# Autodesk Inventor assembly: Drivebase AM14U4 Square 28inx28in v41
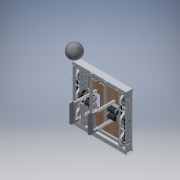
[picture p0: Inventor's stored thumbnail of the model, 180x180]
Saved by Autodesk Inventor 2018 (Build 220112000, 112)
## iProperties
Created: 2020-01-28
Part Number: Drivebase AM14U4 Square 28inx28in v41
Document SubType Name: Assembly
Designer: Weeb No1
Sending System: Autodesk Translation Framework v8.12.0.6
Preprocessor: ST-DEVELOPER v18
Title: /Users/GabG/Documents/GitHub/2020CAD/New Gabriel Shooter/Drivebase AM14U4 Square 28inx28in v41.step
## Documents named in this file (18)
- C:\Users\Weeb No1\Documents\GitHub\2020CAD\New Gabriel Shooter\Main Assembly Files\Drivebase AM14U4 Square 28inx28in v41.iam
- C:\Users\Weeb No1\Documents\GitHub\2020CAD\New Gabriel Shooter\Main Assembly Files\AM14U4 Square Half.iam
- C:\Users\Weeb No1\Documents\GitHub\2020CAD\New Gabriel Shooter\Main Assembly Files\AM14U4 Square Half_1.iam
- C:\Users\Weeb No1\Documents\GitHub\2020CAD\New Gabriel Shooter\Main Assembly Files\Placeholder Belly Pan.ipt
- C:\Users\Weeb No1\Documents\GitHub\2020CAD\New Gabriel Shooter\Main Assembly Files\10-24 Washer.ipt
- C:\Users\Weeb No1\Documents\GitHub\2020CAD\New Gabriel Shooter\Main Assembly Files\Bumper Assembly.iam
- C:\Users\Weeb No1\Documents\GitHub\2020CAD\New Gabriel Shooter\Main Assembly Files\Bumper Assembly_1.iam
- C:\Users\Weeb No1\Documents\GitHub\2020CAD\New Gabriel Shooter\Main Assembly Files\95335A503_METRIC QUICK-RELEASE PIN.ipt
- C:\Users\Weeb No1\Documents\GitHub\2020CAD\New Gabriel Shooter\Main Assembly Files\8020 1010 x 19 v2.ipt
- C:\Users\Weeb No1\Documents\GitHub\2020CAD\New Gabriel Shooter\Main Assembly Files\8020 1010 x 11 5 v2.ipt
- C:\Users\Weeb No1\Documents\GitHub\2020CAD\New Gabriel Shooter\Main Assembly Files\1x2 9in 1_16_ Beam v7.ipt
- C:\Users\Weeb No1\Documents\GitHub\2020CAD\New Gabriel Shooter\Main Assembly Files\L-Guesset v1.ipt
- C:\Users\Weeb No1\Documents\GitHub\2020CAD\New Gabriel Shooter\Main Assembly Files\L-Bracket v1.ipt
- C:\Users\Weeb No1\Documents\GitHub\2020CAD\New Gabriel Shooter\Main Assembly Files\Component52.ipt
- C:\Users\Weeb No1\Documents\GitHub\2020CAD\New Gabriel Shooter\Main Assembly Files\8020 1010 x 8 7_8 v6.ipt
- C:\Users\Weeb No1\Documents\GitHub\2020CAD\New Gabriel Shooter\Main Assembly Files\am-2986 FR8ZZ Hex Bearing v1.ipt
- C:\Users\Weeb No1\Documents\GitHub\2020CAD\New Gabriel Shooter\Main Assembly Files\Clamping_Shaft_Collar_-_1_2_Hex_ID_217-2737 v1.ipt
- C:\Users\Weeb No1\Documents\GitHub\2020CAD\New Gabriel Shooter\Main Assembly Files\1_16_Acetal_Spacer_-_1_2_Hex_217-3257 v1.ipt
## Components (60 placed, 15 different names)
1. AM14U4 Square Half:1 [sub-assembly] — Flush:1, Flush:2, Mate:1, Flush:3, Flush:4, Mate:2
2. AM14U4 Square Half:2 [sub-assembly]
3. Placeholder Belly Pan:1 — Mate:21, Mate:22
4. 10-24 Washer:1
5. 10-24 Washer:2
6. 10-24 Washer:3
7. 10-24 Washer:4
8. 10-24 Washer:5
9. 10-24 Washer:6
10. 10-24 Washer:7
11. 10-24 Washer:8
12. Bumper Assembly:1 [sub-assembly]
13. Bumper Assembly:2 [sub-assembly]
14. 95335A503_METRIC QUICK-RELEASE PIN:1
15. 95335A503_METRIC QUICK-RELEASE PIN:2
16. 95335A503_METRIC QUICK-RELEASE PIN:3
17. 95335A503_METRIC QUICK-RELEASE PIN:4
18. 95335A503_METRIC QUICK-RELEASE PIN:5
19. 95335A503_METRIC QUICK-RELEASE PIN:6
20. 95335A503_METRIC QUICK-RELEASE PIN:7
21. 95335A503_METRIC QUICK-RELEASE PIN:8
22. 95335A503_METRIC QUICK-RELEASE PIN:9
23. 95335A503_METRIC QUICK-RELEASE PIN:10
24. 95335A503_METRIC QUICK-RELEASE PIN:11
25. 95335A503_METRIC QUICK-RELEASE PIN:12
26. 8020 1010 x 19 v2:1 — Flush:1, Flush:2, Mate:1, Mate:19, Mate:20, Flush:17
27. 8020 1010 x 19 v2:2 — Flush:3, Flush:4, Mate:2
28. 8020 1010 x 11 5 v2:1 — Flush:15, Flush:16, Mate:18, Mate:20, Flush:17, Mate:21, Mate:25, Flush:18
29. 8020 1010 x 11 5 v2:2
30. 8020 1010 x 11 5 v2:3 — Mate:17, Flush:13, Flush:14, Mate:19, Mate:22, Mate:29, Flush:21
31. 1x2 9in 1/16" Beam v7:1 — Flush:5, Flush:6, Mate:3, Mate:4, Mate:5, Flush:7, Flush:8, Mate:6, Mate:7, Mate:8, Flush:9, Flush:10, Mate:9, Mate:10, Mate:11, Flush:11, Flush:12, Mate:12, Mate:13, Mate:14, Mate:15, Mate:16, Mate:17, Flush:13, Flush:14, Flush:15, Flush:16, Mate:18
32. 8020 1010 x 11 5 v2:4
33. 1x2 9in 1/16" Beam v7:2
34. L-Guesset v1:1 — Mate:23, Mate:24, Mate:25, Flush:18, Mate:26, Mate:27, Flush:19
35. L-Bracket v1:1 — Mate:26, Mate:27, Mate:28, Flush:19, Flush:20
36. L-Guesset v1:2
37. L-Bracket v1:2
38. L-Guesset v1:3 — Flush:7, Flush:8, Mate:6, Mate:7, Mate:8
39. L-Guesset v1:4 — Flush:11, Flush:12, Mate:12, Mate:13, Mate:14
40. L-Guesset v1:5
41. L-Guesset v1:6
42. L-Guesset v1:7 — Flush:5, Flush:6, Mate:3, Mate:4, Mate:5
43. L-Guesset v1:8 — Flush:9, Flush:10, Mate:9, Mate:10, Mate:11
44. L-Guesset v1:9
45. L-Guesset v1:10
46. L-Bracket v1:3
47. L-Bracket v1:4
48. Component52:1
49. L-Guesset v1:11 — Mate:29, Mate:30, Mate:31, Flush:21, Flush:22
50. L-Guesset v1:12
51. L-Bracket v1:5
52. L-Bracket v1:6
53. L-Bracket v1:7
54. L-Bracket v1:8
55. 8020 1010 x 8 7_8 v6:1
56. 8020 1010 x 8 7_8 v6:2 — Mate:23, Mate:24, Mate:28, Flush:20, Mate:30, Mate:31, Flush:22
57. am-2986 FR8ZZ Hex Bearing v1:1
58. Clamping_Shaft_Collar_-_1_2_Hex_ID_217-2737 v1:1
59. am-2986 FR8ZZ Hex Bearing v1:2 — Mate:15, Mate:16
60. 1_16_Acetal_Spacer_-_1_2_Hex_217-3257 v1:1
## Relationships (53: Mate 31, Flush 22)
- Flush:1: AM14U4 Square Half:1 ↔ 8020 1010 x 19 v2:1
- Flush:2 (247.65 mm): AM14U4 Square Half:1 ↔ 8020 1010 x 19 v2:1
- Mate:1: AM14U4 Square Half:1 ↔ 8020 1010 x 19 v2:1
- Flush:3: AM14U4 Square Half:1 ↔ 8020 1010 x 19 v2:2
- Flush:4 (247.65 mm): AM14U4 Square Half:1 ↔ 8020 1010 x 19 v2:2
- Mate:2: AM14U4 Square Half:1 ↔ 8020 1010 x 19 v2:2
- Flush:5: 1x2 9in 1/16" Beam v7:1 ↔ L-Guesset v1:7
- Flush:6: 1x2 9in 1/16" Beam v7:1 ↔ L-Guesset v1:7
- Mate:3: 1x2 9in 1/16" Beam v7:1 ↔ L-Guesset v1:7
- Mate:4: 1x2 9in 1/16" Beam v7:1 ↔ L-Guesset v1:7
- Mate:5: 1x2 9in 1/16" Beam v7:1 ↔ L-Guesset v1:7
- Flush:7: 1x2 9in 1/16" Beam v7:1 ↔ L-Guesset v1:3
- Flush:8: 1x2 9in 1/16" Beam v7:1 ↔ L-Guesset v1:3
- Mate:6: 1x2 9in 1/16" Beam v7:1 ↔ L-Guesset v1:3
- Mate:7: 1x2 9in 1/16" Beam v7:1 ↔ L-Guesset v1:3
- Mate:8: 1x2 9in 1/16" Beam v7:1 ↔ L-Guesset v1:3
- Flush:9: 1x2 9in 1/16" Beam v7:1 ↔ L-Guesset v1:8
- Flush:10: 1x2 9in 1/16" Beam v7:1 ↔ L-Guesset v1:8
- Mate:9: 1x2 9in 1/16" Beam v7:1 ↔ L-Guesset v1:8
- Mate:10: 1x2 9in 1/16" Beam v7:1 ↔ L-Guesset v1:8
- Mate:11: 1x2 9in 1/16" Beam v7:1 ↔ L-Guesset v1:8
- Flush:11: 1x2 9in 1/16" Beam v7:1 ↔ L-Guesset v1:4
- Flush:12: 1x2 9in 1/16" Beam v7:1 ↔ L-Guesset v1:4
- Mate:12: 1x2 9in 1/16" Beam v7:1 ↔ L-Guesset v1:4
- Mate:13: 1x2 9in 1/16" Beam v7:1 ↔ L-Guesset v1:4
- Mate:14: 1x2 9in 1/16" Beam v7:1 ↔ L-Guesset v1:4
- Mate:15: 1x2 9in 1/16" Beam v7:1 ↔ am-2986 FR8ZZ Hex Bearing v1:2
- Mate:16: 1x2 9in 1/16" Beam v7:1 ↔ am-2986 FR8ZZ Hex Bearing v1:2
- Mate:17: 8020 1010 x 11 5 v2:3 ↔ 1x2 9in 1/16" Beam v7:1
- Flush:13: 8020 1010 x 11 5 v2:3 ↔ 1x2 9in 1/16" Beam v7:1
- Flush:14: 8020 1010 x 11 5 v2:3 ↔ 1x2 9in 1/16" Beam v7:1
- Flush:15: 8020 1010 x 11 5 v2:1 ↔ 1x2 9in 1/16" Beam v7:1
- Flush:16: 8020 1010 x 11 5 v2:1 ↔ 1x2 9in 1/16" Beam v7:1
- Mate:18: 8020 1010 x 11 5 v2:1 ↔ 1x2 9in 1/16" Beam v7:1
- Mate:19: 8020 1010 x 19 v2:1 ↔ 8020 1010 x 11 5 v2:3
- Mate:20: 8020 1010 x 19 v2:1 ↔ 8020 1010 x 11 5 v2:1
- Flush:17 (9.525 mm): 8020 1010 x 19 v2:1 ↔ 8020 1010 x 11 5 v2:1
- Mate:21: Placeholder Belly Pan:1 ↔ 8020 1010 x 11 5 v2:1
- Mate:22: Placeholder Belly Pan:1 ↔ 8020 1010 x 11 5 v2:3
- Mate:23: L-Guesset v1:1 ↔ 8020 1010 x 8 7_8 v6:2
- Mate:24: L-Guesset v1:1 ↔ 8020 1010 x 8 7_8 v6:2
- Mate:25: 8020 1010 x 11 5 v2:1 ↔ L-Guesset v1:1
- Flush:18: 8020 1010 x 11 5 v2:1 ↔ L-Guesset v1:1
- Mate:26: L-Guesset v1:1 ↔ L-Bracket v1:1
- Mate:27: L-Guesset v1:1 ↔ L-Bracket v1:1
- Mate:28: L-Bracket v1:1 ↔ 8020 1010 x 8 7_8 v6:2
- Flush:19: L-Guesset v1:1 ↔ L-Bracket v1:1
- Flush:20: L-Bracket v1:1 ↔ 8020 1010 x 8 7_8 v6:2
- Mate:29: 8020 1010 x 11 5 v2:3 ↔ L-Guesset v1:11
- Mate:30: L-Guesset v1:11 ↔ 8020 1010 x 8 7_8 v6:2
- Mate:31: L-Guesset v1:11 ↔ 8020 1010 x 8 7_8 v6:2
- Flush:21: 8020 1010 x 11 5 v2:3 ↔ L-Guesset v1:11
- Flush:22: L-Guesset v1:11 ↔ 8020 1010 x 8 7_8 v6:2
